# Autodesk Inventor assembly: ThrusterAssembly
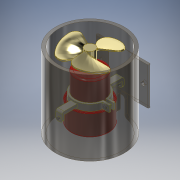
[picture p0: Inventor's stored thumbnail of the model, 180x180]
Saved by Autodesk Inventor 2019 (Build 230136000, 136)
## iProperties
Created: 2019-03-02
Part Number: ThrusterAssembly
Document SubType Name: Assembly
Designer: User
Author: User
## Documents named in this file (8)
- W:\CHAR NOTES\PROJECT\WORKING DRAWINGS\ThrusterAssembly.iam
- W:\CHAR NOTES\PROJECT\WORKING DRAWINGS\SupportBracket_v2_BilgePumpMotor.ipt
- W:\CHAR NOTES\PROJECT\WORKING DRAWINGS\Rear Thruster 2.0.ipt
- C:\Users\User\Documents\Inventor\Content Center Files\R2019\en-US\BS EN 24 036\BS EN 24 036 - M3.5 _.ipt
- W:\CHAR NOTES\PROJECT\WORKING DRAWINGS\Propeller Shroud.ipt
- C:\Users\User\Documents\Inventor\Content Center Files\R2019\en-US\SS-ISO 1207\ISO 1207 - M3.5 x 6SS-ISO.ipt
- C:\Users\User\Documents\Inventor\Content Center Files\R2019\en-US\DIN 923\DIN 923 - M3 x 8.ipt
- W:\CHAR NOTES\PROJECT\WORKING DRAWINGS\Bilge-pump-motor.ipt
## Components (8 placed, 7 different names)
1. SupportBracket_v2_BilgePumpMotor:1 — Insert:1, Insert:2, Insert:3, Insert:5, Insert:6
2. Bilge-pump-motor:1 — Insert:1, Rigid:1, Insert:4
3. Rear Thruster 2.0:1 — Rigid:1
4. DIN 923 M3 x 8:1 — Insert:2
5. BS EN 24036 M3.5 *:1 — Insert:3
6. Propeller Shroud:1 — Insert:4
7. SS ISO 1207 M3.5 x 6:1 — Insert:5
8. SS ISO 1207 M3.5 x 6:2 — Insert:6
## Relationships (7: Insert 6, WeldJoint 1)
- Insert:1 (-29 mm): SupportBracket_v2_BilgePumpMotor:1 ↔ Bilge-pump-motor:1
- Rigid:1 [WeldJoint]: Bilge-pump-motor:1 ↔ Rear Thruster 2.0:1
- Insert:2: SupportBracket_v2_BilgePumpMotor:1 ↔ DIN 923 M3 x 8:1
- Insert:3: SupportBracket_v2_BilgePumpMotor:1 ↔ BS EN 24036 M3.5 *:1
- Insert:4 (-72 mm): Bilge-pump-motor:1 ↔ Propeller Shroud:1
- Insert:5: SupportBracket_v2_BilgePumpMotor:1 ↔ SS ISO 1207 M3.5 x 6:1
- Insert:6: SupportBracket_v2_BilgePumpMotor:1 ↔ SS ISO 1207 M3.5 x 6:2
